# Autodesk Inventor assembly: newkrablerus
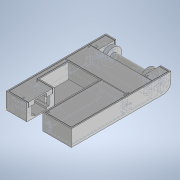
[picture p0: Inventor's stored thumbnail of the model, 180x180]
Saved by Autodesk Inventor 2020 (Build 240168000, 168)
## iProperties
Created: 2021-01-11
Part Number: newkrablerus
Document SubType Name: Assembly
Designer: papa
Author: papa
## Documents named in this file (9)
- C:\Users\papa\Documents\Inventor\newkrablerus\newkrablerus.iam
- C:\Users\papa\Documents\Inventor\newkrablerus\batteryholder.ipt
- C:\Users\papa\Documents\Inventor\newkrablerus\bearingholder.ipt
- C:\Users\papa\Documents\Inventor\newkrablerus\body.ipt
- C:\Users\papa\Documents\Inventor\newkrablerus\brainholder.ipt
- C:\Users\papa\Documents\Inventor\newkrablerus\encoderholder.ipt
- C:\Users\papa\Documents\Inventor\newkrablerus\servoholder.ipt
- C:\Users\papa\Documents\Inventor\newkrablerus\wheelaxis.ipt
- C:\Users\papa\Documents\Inventor\newkrablerus\secondwheel.ipt
## Components (8 placed, 8 different names)
1. batteryholder:1 — Mate:1, Mate:2
2. bearingholder:1 — Mate:6, Flush:1
3. body:1 — Mate:1, Mate:2, Mate:3, Mate:4, Mate:5, Mate:6, Flush:1, Flush:2, Mate:7, Mate:8, Mate:11
4. brainholder:1 — Mate:3, Mate:4
5. encoderholder:1 — Mate:5, Flush:2
6. servoholder:1 — Mate:7, Mate:8
7. wheelaxis:1 — Mate:9, Mate:10, Mate:11
8. secondwheel:1 — Mate:9, Mate:10
## Relationships (13: Mate 11, Flush 2)
- Mate:1: batteryholder:1 ↔ body:1
- Mate:2: batteryholder:1 ↔ body:1
- Mate:3: body:1 ↔ brainholder:1
- Mate:4: body:1 ↔ brainholder:1
- Mate:5: body:1 ↔ encoderholder:1
- Mate:6: bearingholder:1 ↔ body:1
- Flush:1: bearingholder:1 ↔ body:1
- Flush:2: body:1 ↔ encoderholder:1
- Mate:7: body:1 ↔ servoholder:1
- Mate:8: body:1 ↔ servoholder:1
- Mate:9: wheelaxis:1 ↔ secondwheel:1
- Mate:10: wheelaxis:1 ↔ secondwheel:1
- Mate:11: body:1 ↔ wheelaxis:1
